# Autodesk Inventor assembly: Digital Loggers IoT Relay
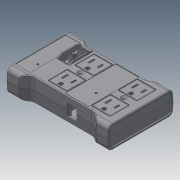
[picture p0: Inventor's stored thumbnail of the model, 180x180]
Saved by Autodesk Inventor 2020.3 (Build 243373000, 373)
## iProperties
RuleStatus: InUse
AfterDocSave0: file://Part Number Cleaner
Created: 2023-02-09
Catalog Web Link: https://www.janelia.org/
Vendor: HHMI: JRC - jET
Document SubType Name: Assembly
Designer: arnoldj
DESIGN DEPARTMENT: HHMI: JRC - jET
ALTERED ITEM PART NUMBER: N/A
ALTERED ITEM VENDOR: N/A
ALTERED ITEM DESCRIPTION: N/A
PART NUMBER - LEGACY: Standard
Author: arnoldj
Revision Number: 0
## Documents named in this file (5)
- C:\_WORKSPACE\DATA\COMMON\Digital Loggers\Digital Loggers IoT Relay.iam
- C:\_WORKSPACE\DATA\COMMON\Digital Loggers\Digital Loggers IoT Relay Bottom.ipt
- C:\_WORKSPACE\DATA\COMMON\Digital Loggers\Digital Loggers IoT Relay Top.ipt
- C:\_WORKSPACE\DATA\COMMON\McMaster\MCMASTER 1333N19.ipt
- C:\_WORKSPACE\DATA\COMMON\McMaster\MCMASTER 7168K1.ipt
## Components (7 placed, 4 different names)
1. Digital Loggers IoT Relay Bottom:1 — Mate:7, Mate:8, Mate:9
2. Digital Loggers IoT Relay Top:1 — Flush:2, Flush:3, Mate:5, Mate:7, Mate:8, Mate:9, Mate:10, Mate:11
3. MCMASTER 1333N19:1 — Flush:2, Flush:5, Mate:11
4. MCMASTER 7168K1:1 — Flush:3, Mate:5, Mate:10
5. MCMASTER 7168K1:2
6. MCMASTER 7168K1:3
7. MCMASTER 7168K1:4
## Component patterns: (4 elements, first: MCMASTER 7168K1:1)
## Relationships (9: Mate 6, Flush 3)
- Flush:2: Digital Loggers IoT Relay Top:1 ↔ MCMASTER 1333N19:1
- Flush:5: MCMASTER 1333N19:1
- Flush:3: Digital Loggers IoT Relay Top:1 ↔ MCMASTER 7168K1:1
- Mate:5 (0.508 mm): Digital Loggers IoT Relay Top:1 ↔ MCMASTER 7168K1:1
- Mate:7: Digital Loggers IoT Relay Bottom:1 ↔ Digital Loggers IoT Relay Top:1
- Mate:8: Digital Loggers IoT Relay Bottom:1 ↔ Digital Loggers IoT Relay Top:1
- Mate:9: Digital Loggers IoT Relay Bottom:1 ↔ Digital Loggers IoT Relay Top:1
- Mate:10 (1.27 mm): Digital Loggers IoT Relay Top:1 ↔ MCMASTER 7168K1:1
- Mate:11 (-6.35 mm): Digital Loggers IoT Relay Top:1 ↔ MCMASTER 1333N19:1
